# Autodesk Inventor assembly: KB33-046-008 - Блок АКБ
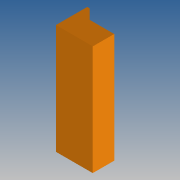
[picture p0: Inventor's stored thumbnail of the model, 180x180]
Saved by Autodesk Inventor 2020 (Build 240168000, 168)
## iProperties
Created: 2021-08-09
Part Number: KB33-046-008 - Блок АКБ
Document SubType Name: Assembly
Designer: Петров Иван
Mass: 423.528 g
Surface Area: 1147.15 cm^2
Volume: 423.528 cm^3
Density: 1 g/cm^3
Author: Петров Иван
## Documents named in this file (3)
- C:\Users\Ivan\Documents\GitHub\RoboPatrol\design\KB33-046-008 - Блок АКБ.iam
- C:\Users\Ivan\Documents\GitHub\RoboPatrol\design\KB33-046-008-001 - Корпус.ipt
- C:\Users\Ivan\Documents\GitHub\RoboPatrol\design\standart_components\Turnigy 4S 5200 mah\Turnigy 4S 5200 mah.ipt
## Components (2 placed, 2 different names)
1. KB33-046-008-001 - Корпус:1 — Совмещение:2, Совмещение:3, Совмещение:4
2. Turnigy 4S 5200 mah:1 — Совмещение:2, Совмещение:3, Совмещение:4
## Relationships (3: Mate 3)
- Совмещение:2 [Mate]: KB33-046-008-001 - Корпус:1 ↔ Turnigy 4S 5200 mah:1
- Совмещение:3 [Mate]: KB33-046-008-001 - Корпус:1 ↔ Turnigy 4S 5200 mah:1
- Совмещение:4 [Mate]: KB33-046-008-001 - Корпус:1 ↔ Turnigy 4S 5200 mah:1
